# Autodesk Inventor assembly: VerticalBit
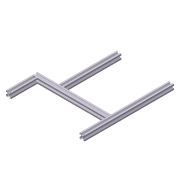
[picture p0: Inventor's stored thumbnail of the model, 180x180]
Saved by Autodesk Inventor 2014 (Build 180170000, 170)
## iProperties
Created: 2014-08-09
Part Number: VerticalBit
Document SubType Name: Assembly
Designer: Peele
Author: Peele
## Documents named in this file (6)
- E:\Copy\DLP\PandaPrint\SubAssem\VerticalBit.iam
- E:\Copy\DLP\PandaPrint\StockParts\8020-25\8020-2515.ipt
- E:\Copy\DLP\PandaPrint\StockParts\8020-25\8020-2516.ipt
- E:\Copy\DLP\PandaPrint\StockParts\8020-25.ipt
- E:\Copy\DLP\PandaPrint\StockParts\8020-25\8020-2510.ipt
- E:\Copy\DLP\PandaPrint\StockParts\8020-25\8020-2519.ipt
## Components (4 placed, 4 different names)
1. 8020-2515:5 — Mate:9, Mate:10, Flush:11
2. 8020-2516:3 — Mate:6, Flush:7, Mate:9, Flush:10
3. 8020-2510:6 — Mate:6, Flush:7, Mate:8, Flush:8, Flush:9, Mate:10, Flush:11
4. 8020-2519:8 — Mate:8, Flush:8, Flush:9, Flush:10
## Relationships (9: Flush 5, Mate 4)
- Mate:6: 8020-2516:3 ↔ 8020-2510:6
- Flush:7: 8020-2516:3 ↔ 8020-2510:6
- Mate:8: 8020-2510:6 ↔ 8020-2519:8
- Flush:8: 8020-2510:6 ↔ 8020-2519:8
- Flush:9: 8020-2510:6 ↔ 8020-2519:8
- Mate:9 (225 mm): 8020-2515:5 ↔ 8020-2516:3
- Flush:10: 8020-2516:3 ↔ 8020-2519:8
- Mate:10: 8020-2515:5 ↔ 8020-2510:6
- Flush:11: 8020-2515:5 ↔ 8020-2510:6
